# Autodesk Inventor assembly: 110033226_iam_07_中心城堡.iiam
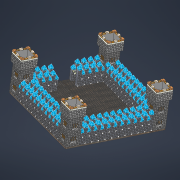
[picture p0: Inventor's stored thumbnail of the model, 180x180]
Saved by Autodesk Inventor 2022 (Build 260153000, 153)
## iProperties
Created: 2022-06-24
Part Number: 110033226_iam_07_中心城堡.iiam
Document SubType Name: Assembly
Designer: User
Author: User
## Documents named in this file (6)
- D:\D-disk\pomelo\大一\下學期\機械設計製圖\1100332260_LEGOproj_沒有公主城堡\110033226_iam_07_中心城堡.iiam.iam
- D:\D-disk\pomelo\大一\下學期\機械設計製圖\1100332260_LEGOproj_沒有公主城堡\110033226_ipt_33_中心城堡基座.ipt
- D:\D-disk\pomelo\大一\下學期\機械設計製圖\1100332260_LEGOproj_沒有公主城堡\110033226_iam_06_城堡四角塔.iam
- D:\D-disk\pomelo\大一\下學期\機械設計製圖\1100332260_LEGOproj_沒有公主城堡\110033226_ipt_34_中心城堡圍牆.ipt
- D:\D-disk\pomelo\大一\下學期\機械設計製圖\1100332260_LEGOproj_沒有公主城堡\110033226_ipt_34_中心城堡圍牆_MIR.ipt
- D:\D-disk\pomelo\大一\下學期\機械設計製圖\1100332260_LEGOproj_沒有公主城堡\110033226_ipt_35_中心城堡圍牆頂部_MIR.ipt
## Components (251 placed, 5 different names)
1. 110033226_ipt_33_中心城堡基座:1 — 貼合:1, 貼合:2, 貼合:3, 貼合:4, 貼合:5, 貼合:6, 貼合:7, 貼合:8, 貼合:9, 貼合:10, 貼合:11, 貼合:12, 貼合:24, 貼合:25, 貼合:26, 貼合:27, 貼合:29
2. 110033226_iam_06_城堡四角塔:1 [sub-assembly] — 貼合:4, 貼合:5, 貼合:6
3. 110033226_iam_06_城堡四角塔:2 [sub-assembly]
4. 110033226_iam_06_城堡四角塔:3 [sub-assembly]
5. 110033226_iam_06_城堡四角塔:4 [sub-assembly]
6. 110033226_ipt_34_中心城堡圍牆_MIR:1 — 貼合:10, 貼合:11, 貼合:12, 貼合:13, 貼合:14, 貼合:15, 貼合:16, 貼合:17
7. 110033226_ipt_34_中心城堡圍牆_MIR:2
8. 110033226_ipt_34_中心城堡圍牆_MIR:3
9. 110033226_ipt_34_中心城堡圍牆_MIR:4
10. 110033226_ipt_34_中心城堡圍牆_MIR:5
11. 110033226_ipt_34_中心城堡圍牆_MIR:6
12. 110033226_ipt_34_中心城堡圍牆_MIR:7
13. 110033226_ipt_34_中心城堡圍牆_MIR:8
14. 110033226_ipt_34_中心城堡圍牆_MIR:9
15. 110033226_ipt_34_中心城堡圍牆_MIR:10
16. 110033226_ipt_34_中心城堡圍牆_MIR:11
17. 110033226_ipt_34_中心城堡圍牆:1 — 貼合:7, 貼合:8, 貼合:9, 貼合:18, 貼合:19, 貼合:20, 貼合:21, 貼合:22, 貼合:23
18. 110033226_ipt_34_中心城堡圍牆:2
19. 110033226_ipt_34_中心城堡圍牆:3
20. 110033226_ipt_34_中心城堡圍牆:4
21. 110033226_ipt_34_中心城堡圍牆:5
22. 110033226_ipt_34_中心城堡圍牆:6
23. 110033226_ipt_34_中心城堡圍牆:7
24. 110033226_ipt_34_中心城堡圍牆:8
25. 110033226_ipt_34_中心城堡圍牆:9
26. 110033226_ipt_34_中心城堡圍牆:10
27. 110033226_ipt_34_中心城堡圍牆:11
28. 110033226_ipt_34_中心城堡圍牆_MIR:12
29. 110033226_ipt_34_中心城堡圍牆_MIR:13
30. 110033226_ipt_34_中心城堡圍牆_MIR:14
31. 110033226_ipt_34_中心城堡圍牆_MIR:15
32. 110033226_ipt_34_中心城堡圍牆_MIR:16
33. 110033226_ipt_34_中心城堡圍牆_MIR:17
34. 110033226_ipt_34_中心城堡圍牆_MIR:18
35. 110033226_ipt_34_中心城堡圍牆_MIR:19
36. 110033226_ipt_34_中心城堡圍牆_MIR:20
37. 110033226_ipt_34_中心城堡圍牆_MIR:21
38. 110033226_ipt_34_中心城堡圍牆_MIR:22
39. 110033226_ipt_34_中心城堡圍牆:12
40. 110033226_ipt_34_中心城堡圍牆:13
41. 110033226_ipt_34_中心城堡圍牆:14
42. 110033226_ipt_34_中心城堡圍牆:15
43. 110033226_ipt_34_中心城堡圍牆:16
44. 110033226_ipt_34_中心城堡圍牆:17
45. 110033226_ipt_34_中心城堡圍牆:18
46. 110033226_ipt_34_中心城堡圍牆:19
47. 110033226_ipt_34_中心城堡圍牆:20
48. 110033226_ipt_34_中心城堡圍牆:21
49. 110033226_ipt_34_中心城堡圍牆:22
50. 110033226_ipt_34_中心城堡圍牆_MIR:23
51. 110033226_ipt_34_中心城堡圍牆_MIR:24
52. 110033226_ipt_34_中心城堡圍牆_MIR:25
53. 110033226_ipt_34_中心城堡圍牆_MIR:26
54. 110033226_ipt_34_中心城堡圍牆_MIR:27
55. 110033226_ipt_34_中心城堡圍牆_MIR:28
56. 110033226_ipt_34_中心城堡圍牆_MIR:29
57. 110033226_ipt_34_中心城堡圍牆_MIR:30
58. 110033226_ipt_34_中心城堡圍牆_MIR:31
59. 110033226_ipt_34_中心城堡圍牆_MIR:32
60. 110033226_ipt_34_中心城堡圍牆_MIR:33
61. 110033226_ipt_34_中心城堡圍牆:23
62. 110033226_ipt_34_中心城堡圍牆:24
63. 110033226_ipt_34_中心城堡圍牆:25
64. 110033226_ipt_34_中心城堡圍牆:26
65. 110033226_ipt_34_中心城堡圍牆:27
66. 110033226_ipt_34_中心城堡圍牆:28
67. 110033226_ipt_34_中心城堡圍牆:29
68. 110033226_ipt_34_中心城堡圍牆:30
69. 110033226_ipt_34_中心城堡圍牆:31
70. 110033226_ipt_34_中心城堡圍牆:32
71. 110033226_ipt_34_中心城堡圍牆:33
72. 110033226_ipt_35_中心城堡圍牆頂部_MIR:3 — 貼合:16, 貼合:17
73. 110033226_ipt_35_中心城堡圍牆頂部_MIR:4 — 貼合:13, 貼合:14, 貼合:15
74. 110033226_ipt_35_中心城堡圍牆頂部_MIR:1 — 貼合:21, 貼合:22, 貼合:23
75. 110033226_ipt_35_中心城堡圍牆頂部_MIR:2 — 貼合:18, 貼合:19, 貼合:20
76. 110033226_ipt_35_中心城堡圍牆頂部_MIR:5
77. 110033226_ipt_35_中心城堡圍牆頂部_MIR:6
78. 110033226_ipt_35_中心城堡圍牆頂部_MIR:7
79. 110033226_ipt_35_中心城堡圍牆頂部_MIR:8
80. 110033226_ipt_35_中心城堡圍牆頂部_MIR:9
81. 110033226_ipt_35_中心城堡圍牆頂部_MIR:10
82. 110033226_ipt_35_中心城堡圍牆頂部_MIR:11
83. 110033226_ipt_35_中心城堡圍牆頂部_MIR:12
84. 110033226_ipt_35_中心城堡圍牆頂部_MIR:13
85. 110033226_ipt_35_中心城堡圍牆頂部_MIR:14
86. 110033226_ipt_35_中心城堡圍牆頂部_MIR:15
87. 110033226_ipt_35_中心城堡圍牆頂部_MIR:16
88. 110033226_ipt_35_中心城堡圍牆頂部_MIR:17
89. 110033226_ipt_35_中心城堡圍牆頂部_MIR:18
90. 110033226_ipt_35_中心城堡圍牆頂部_MIR:19
91. 110033226_ipt_35_中心城堡圍牆頂部_MIR:20
92. 110033226_ipt_35_中心城堡圍牆頂部_MIR:21
93. 110033226_ipt_35_中心城堡圍牆頂部_MIR:22
94. 110033226_ipt_35_中心城堡圍牆頂部_MIR:23
95. 110033226_ipt_35_中心城堡圍牆頂部_MIR:24
96. 110033226_ipt_35_中心城堡圍牆頂部_MIR:25
97. 110033226_ipt_35_中心城堡圍牆頂部_MIR:26
98. 110033226_ipt_35_中心城堡圍牆頂部_MIR:27
99. 110033226_ipt_35_中心城堡圍牆頂部_MIR:28
100. 110033226_ipt_35_中心城堡圍牆頂部_MIR:29
101. 110033226_ipt_35_中心城堡圍牆頂部_MIR:30
102. 110033226_ipt_35_中心城堡圍牆頂部_MIR:31
103. 110033226_ipt_35_中心城堡圍牆頂部_MIR:32
104. 110033226_ipt_35_中心城堡圍牆頂部_MIR:33
105. 110033226_ipt_35_中心城堡圍牆頂部_MIR:34
106. 110033226_ipt_35_中心城堡圍牆頂部_MIR:35
107. 110033226_ipt_35_中心城堡圍牆頂部_MIR:36
108. 110033226_ipt_35_中心城堡圍牆頂部_MIR:37
109. 110033226_ipt_35_中心城堡圍牆頂部_MIR:38
110. 110033226_ipt_35_中心城堡圍牆頂部_MIR:39
111. 110033226_ipt_35_中心城堡圍牆頂部_MIR:40
112. 110033226_ipt_35_中心城堡圍牆頂部_MIR:41
113. 110033226_ipt_35_中心城堡圍牆頂部_MIR:42
114. 110033226_ipt_35_中心城堡圍牆頂部_MIR:43
115. 110033226_ipt_35_中心城堡圍牆頂部_MIR:44
116. 110033226_ipt_35_中心城堡圍牆頂部_MIR:45
117. 110033226_ipt_35_中心城堡圍牆頂部_MIR:46
118. 110033226_ipt_35_中心城堡圍牆頂部_MIR:47
119. 110033226_ipt_35_中心城堡圍牆頂部_MIR:48
120. 110033226_ipt_35_中心城堡圍牆頂部_MIR:49
121. 110033226_ipt_35_中心城堡圍牆頂部_MIR:50
122. 110033226_ipt_35_中心城堡圍牆頂部_MIR:51
123. 110033226_ipt_35_中心城堡圍牆頂部_MIR:52
124. 110033226_ipt_35_中心城堡圍牆頂部_MIR:53
125. 110033226_ipt_35_中心城堡圍牆頂部_MIR:54
126. 110033226_ipt_35_中心城堡圍牆頂部_MIR:55
127. 110033226_ipt_35_中心城堡圍牆頂部_MIR:56
128. 110033226_ipt_35_中心城堡圍牆頂部_MIR:57
129. 110033226_ipt_35_中心城堡圍牆頂部_MIR:58
130. 110033226_ipt_35_中心城堡圍牆頂部_MIR:59
131. 110033226_ipt_35_中心城堡圍牆頂部_MIR:60
132. 110033226_ipt_35_中心城堡圍牆頂部_MIR:61
133. 110033226_ipt_35_中心城堡圍牆頂部_MIR:62
134. 110033226_ipt_35_中心城堡圍牆頂部_MIR:63
135. 110033226_ipt_35_中心城堡圍牆頂部_MIR:64
136. 110033226_ipt_35_中心城堡圍牆頂部_MIR:65
137. 110033226_ipt_35_中心城堡圍牆頂部_MIR:66
138. 110033226_ipt_35_中心城堡圍牆頂部_MIR:67
139. 110033226_ipt_35_中心城堡圍牆頂部_MIR:68
140. 110033226_ipt_35_中心城堡圍牆頂部_MIR:69
141. 110033226_ipt_35_中心城堡圍牆頂部_MIR:70
142. 110033226_ipt_35_中心城堡圍牆頂部_MIR:71
143. 110033226_ipt_35_中心城堡圍牆頂部_MIR:72
144. 110033226_ipt_35_中心城堡圍牆頂部_MIR:73
145. 110033226_ipt_35_中心城堡圍牆頂部_MIR:74
146. 110033226_ipt_35_中心城堡圍牆頂部_MIR:75
147. 110033226_ipt_35_中心城堡圍牆頂部_MIR:76
148. 110033226_ipt_35_中心城堡圍牆頂部_MIR:77
149. 110033226_ipt_35_中心城堡圍牆頂部_MIR:78
150. 110033226_ipt_35_中心城堡圍牆頂部_MIR:79
151. 110033226_ipt_35_中心城堡圍牆頂部_MIR:80
152. 110033226_ipt_35_中心城堡圍牆頂部_MIR:81
153. 110033226_ipt_35_中心城堡圍牆頂部_MIR:82
154. 110033226_ipt_35_中心城堡圍牆頂部_MIR:83
155. 110033226_ipt_35_中心城堡圍牆頂部_MIR:84
156. 110033226_ipt_35_中心城堡圍牆頂部_MIR:85
157. 110033226_ipt_35_中心城堡圍牆頂部_MIR:86
158. 110033226_ipt_35_中心城堡圍牆頂部_MIR:87
159. 110033226_ipt_35_中心城堡圍牆頂部_MIR:88
160. 110033226_ipt_35_中心城堡圍牆頂部_MIR:89
161. 110033226_ipt_35_中心城堡圍牆頂部_MIR:90
162. 110033226_ipt_35_中心城堡圍牆頂部_MIR:91
163. 110033226_ipt_35_中心城堡圍牆頂部_MIR:92
164. 110033226_ipt_35_中心城堡圍牆頂部_MIR:93
165. 110033226_ipt_35_中心城堡圍牆頂部_MIR:94
166. 110033226_ipt_35_中心城堡圍牆頂部_MIR:95
167. 110033226_ipt_35_中心城堡圍牆頂部_MIR:96
168. 110033226_ipt_35_中心城堡圍牆頂部_MIR:97
169. 110033226_ipt_35_中心城堡圍牆頂部_MIR:98
170. 110033226_ipt_35_中心城堡圍牆頂部_MIR:99
171. 110033226_ipt_35_中心城堡圍牆頂部_MIR:100
172. 110033226_ipt_35_中心城堡圍牆頂部_MIR:101
173. 110033226_ipt_35_中心城堡圍牆頂部_MIR:102
174. 110033226_ipt_35_中心城堡圍牆頂部_MIR:103
175. 110033226_ipt_35_中心城堡圍牆頂部_MIR:104
176. 110033226_ipt_35_中心城堡圍牆頂部_MIR:105
177. 110033226_ipt_35_中心城堡圍牆頂部_MIR:106
178. 110033226_ipt_35_中心城堡圍牆頂部_MIR:107
179. 110033226_ipt_35_中心城堡圍牆頂部_MIR:108
180. 110033226_ipt_35_中心城堡圍牆頂部_MIR:109
181. 110033226_ipt_35_中心城堡圍牆頂部_MIR:110
182. 110033226_ipt_35_中心城堡圍牆頂部_MIR:111
183. 110033226_ipt_35_中心城堡圍牆頂部_MIR:112
184. 110033226_ipt_35_中心城堡圍牆頂部_MIR:113
185. 110033226_ipt_35_中心城堡圍牆頂部_MIR:114
186. 110033226_ipt_35_中心城堡圍牆頂部_MIR:115
187. 110033226_ipt_35_中心城堡圍牆頂部_MIR:116
188. 110033226_ipt_35_中心城堡圍牆頂部_MIR:117
189. 110033226_ipt_35_中心城堡圍牆頂部_MIR:118
190. 110033226_ipt_35_中心城堡圍牆頂部_MIR:119
191. 110033226_ipt_35_中心城堡圍牆頂部_MIR:120
192. 110033226_ipt_35_中心城堡圍牆頂部_MIR:121
193. 110033226_ipt_35_中心城堡圍牆頂部_MIR:122
194. 110033226_ipt_35_中心城堡圍牆頂部_MIR:123
195. 110033226_ipt_35_中心城堡圍牆頂部_MIR:124
196. 110033226_ipt_35_中心城堡圍牆頂部_MIR:125
197. 110033226_ipt_35_中心城堡圍牆頂部_MIR:126
198. 110033226_ipt_35_中心城堡圍牆頂部_MIR:127
199. 110033226_ipt_35_中心城堡圍牆頂部_MIR:128
200. 110033226_ipt_35_中心城堡圍牆頂部_MIR:129
201. 110033226_ipt_35_中心城堡圍牆頂部_MIR:130
202. 110033226_ipt_35_中心城堡圍牆頂部_MIR:131
203. 110033226_ipt_35_中心城堡圍牆頂部_MIR:132
204. 110033226_ipt_34_中心城堡圍牆_MIR:34 — 貼合:24, 貼合:25, 貼合:26, 貼合:28, 貼合:30, 貼合:31, 貼合:32, 貼合:39, 貼合:40, 貼合:41
205. 110033226_ipt_34_中心城堡圍牆_MIR:35 — 貼合:27, 貼合:28, 貼合:29, 貼合:33, 貼合:34, 貼合:35, 貼合:36, 貼合:37, 貼合:38
206. 110033226_ipt_34_中心城堡圍牆_MIR:36
207. 110033226_ipt_34_中心城堡圍牆_MIR:37
208. 110033226_ipt_34_中心城堡圍牆_MIR:38
209. 110033226_ipt_34_中心城堡圍牆_MIR:39
210. 110033226_ipt_34_中心城堡圍牆_MIR:40
211. 110033226_ipt_34_中心城堡圍牆_MIR:41
212. 110033226_ipt_34_中心城堡圍牆_MIR:42
213. 110033226_ipt_34_中心城堡圍牆_MIR:43
214. 110033226_ipt_34_中心城堡圍牆_MIR:44
215. 110033226_ipt_34_中心城堡圍牆_MIR:45
216. 110033226_ipt_34_中心城堡圍牆_MIR:46
217. 110033226_ipt_34_中心城堡圍牆_MIR:47
218. 110033226_ipt_34_中心城堡圍牆_MIR:48
219. 110033226_ipt_34_中心城堡圍牆_MIR:49
220. 110033226_ipt_35_中心城堡圍牆頂部_MIR:134 — 貼合:33, 貼合:34, 貼合:35
221. 110033226_ipt_35_中心城堡圍牆頂部_MIR:136 — 貼合:36, 貼合:37, 貼合:38
222. 110033226_ipt_35_中心城堡圍牆頂部_MIR:133 — 貼合:30, 貼合:31, 貼合:32
223. 110033226_ipt_35_中心城堡圍牆頂部_MIR:135 — 貼合:39, 貼合:40, 貼合:41
224. 110033226_ipt_35_中心城堡圍牆頂部_MIR:137
225. 110033226_ipt_35_中心城堡圍牆頂部_MIR:138
226. 110033226_ipt_35_中心城堡圍牆頂部_MIR:139
227. 110033226_ipt_35_中心城堡圍牆頂部_MIR:140
228. 110033226_ipt_35_中心城堡圍牆頂部_MIR:141
229. 110033226_ipt_35_中心城堡圍牆頂部_MIR:142
230. 110033226_ipt_35_中心城堡圍牆頂部_MIR:143
231. 110033226_ipt_35_中心城堡圍牆頂部_MIR:144
232. 110033226_ipt_35_中心城堡圍牆頂部_MIR:145
233. 110033226_ipt_35_中心城堡圍牆頂部_MIR:146
234. 110033226_ipt_35_中心城堡圍牆頂部_MIR:147
235. 110033226_ipt_35_中心城堡圍牆頂部_MIR:148
236. 110033226_ipt_35_中心城堡圍牆頂部_MIR:149
237. 110033226_ipt_35_中心城堡圍牆頂部_MIR:150
238. 110033226_ipt_35_中心城堡圍牆頂部_MIR:151
239. 110033226_ipt_35_中心城堡圍牆頂部_MIR:152
240. 110033226_ipt_35_中心城堡圍牆頂部_MIR:153
241. 110033226_ipt_35_中心城堡圍牆頂部_MIR:154
242. 110033226_ipt_35_中心城堡圍牆頂部_MIR:155
243. 110033226_ipt_35_中心城堡圍牆頂部_MIR:156
244. 110033226_ipt_35_中心城堡圍牆頂部_MIR:157
245. 110033226_ipt_35_中心城堡圍牆頂部_MIR:158
246. 110033226_ipt_35_中心城堡圍牆頂部_MIR:159
247. 110033226_ipt_35_中心城堡圍牆頂部_MIR:160
248. 110033226_ipt_35_中心城堡圍牆頂部_MIR:161
249. 110033226_ipt_35_中心城堡圍牆頂部_MIR:162
250. 110033226_ipt_35_中心城堡圍牆頂部_MIR:163
251. 110033226_ipt_35_中心城堡圍牆頂部_MIR:164
## Component patterns: (4 elements, first: 110033226_iam_06_城堡四角塔:1), (3 elements), (3 elements), (2 elements), (2 elements), (11 elements, first: 110033226_ipt_34_中心城堡圍牆_MIR:1), (11 elements, first: 110033226_ipt_34_中心城堡圍牆:1), 元件陣列 7:2 (11 elements), 元件陣列 4:2 (11 elements), 元件陣列 7:3 (11 elements), 元件陣列 4:3 (11 elements), (11 elements, first: 110033226_ipt_35_中心城堡圍牆頂部_MIR:3 + 110033226_ipt_35_中心城堡圍牆頂部_MIR:4 + 110033226_ipt_35_中心城堡圍牆頂部_MIR:1 + 110033226_ipt_35_中心城堡圍牆頂部_MIR:2), 元件陣列 9:2 (11 elements), 元件陣列 9:3 (11 elements), (4 elements, first: 110033226_ipt_34_中心城堡圍牆_MIR:34 + 110033226_ipt_34_中心城堡圍牆_MIR:35), 元件陣列 11:2 (4 elements), (4 elements, first: 110033226_ipt_35_中心城堡圍牆頂部_MIR:134 + 110033226_ipt_35_中心城堡圍牆頂部_MIR:136 + 110033226_ipt_35_中心城堡圍牆頂部_MIR:133 + 110033226_ipt_35_中心城堡圍牆頂部_MIR:135), 元件陣列 13:2 (4 elements)
## Relationships (41: Mate 41)
- 貼合:1 [Mate]: 110033226_ipt_33_中心城堡基座:1
- 貼合:2 [Mate]: 110033226_ipt_33_中心城堡基座:1
- 貼合:3 [Mate]: 110033226_ipt_33_中心城堡基座:1
- 貼合:4 [Mate]: 110033226_ipt_33_中心城堡基座:1 ↔ 110033226_iam_06_城堡四角塔:1
- 貼合:5 [Mate]: 110033226_ipt_33_中心城堡基座:1 ↔ 110033226_iam_06_城堡四角塔:1
- 貼合:6 [Mate]: 110033226_ipt_33_中心城堡基座:1 ↔ 110033226_iam_06_城堡四角塔:1
- 貼合:7 [Mate]: 110033226_ipt_33_中心城堡基座:1 ↔ 110033226_ipt_34_中心城堡圍牆:1
- 貼合:8 [Mate]: 110033226_ipt_33_中心城堡基座:1 ↔ 110033226_ipt_34_中心城堡圍牆:1
- 貼合:9 [Mate]: 110033226_ipt_33_中心城堡基座:1 ↔ 110033226_ipt_34_中心城堡圍牆:1
- 貼合:10 [Mate]: 110033226_ipt_33_中心城堡基座:1 ↔ 110033226_ipt_34_中心城堡圍牆_MIR:1
- 貼合:11 [Mate]: 110033226_ipt_33_中心城堡基座:1 ↔ 110033226_ipt_34_中心城堡圍牆_MIR:1
- 貼合:12 [Mate]: 110033226_ipt_33_中心城堡基座:1 ↔ 110033226_ipt_34_中心城堡圍牆_MIR:1
- 貼合:13 [Mate]: 110033226_ipt_34_中心城堡圍牆_MIR:1 ↔ 110033226_ipt_35_中心城堡圍牆頂部_MIR:4
- 貼合:14 [Mate]: 110033226_ipt_34_中心城堡圍牆_MIR:1 ↔ 110033226_ipt_35_中心城堡圍牆頂部_MIR:4
- 貼合:15 [Mate]: 110033226_ipt_34_中心城堡圍牆_MIR:1 ↔ 110033226_ipt_35_中心城堡圍牆頂部_MIR:4
- 貼合:16 [Mate]: 110033226_ipt_34_中心城堡圍牆_MIR:1 ↔ 110033226_ipt_35_中心城堡圍牆頂部_MIR:3
- 貼合:17 [Mate]: 110033226_ipt_34_中心城堡圍牆_MIR:1 ↔ 110033226_ipt_35_中心城堡圍牆頂部_MIR:3
- 貼合:18 [Mate]: 110033226_ipt_34_中心城堡圍牆:1 ↔ 110033226_ipt_35_中心城堡圍牆頂部_MIR:2
- 貼合:19 [Mate]: 110033226_ipt_34_中心城堡圍牆:1 ↔ 110033226_ipt_35_中心城堡圍牆頂部_MIR:2
- 貼合:20 [Mate]: 110033226_ipt_34_中心城堡圍牆:1 ↔ 110033226_ipt_35_中心城堡圍牆頂部_MIR:2
- 貼合:21 [Mate]: 110033226_ipt_34_中心城堡圍牆:1 ↔ 110033226_ipt_35_中心城堡圍牆頂部_MIR:1
- 貼合:22 [Mate]: 110033226_ipt_34_中心城堡圍牆:1 ↔ 110033226_ipt_35_中心城堡圍牆頂部_MIR:1
- 貼合:23 [Mate]: 110033226_ipt_34_中心城堡圍牆:1 ↔ 110033226_ipt_35_中心城堡圍牆頂部_MIR:1
- 貼合:24 [Mate]: 110033226_ipt_33_中心城堡基座:1 ↔ 110033226_ipt_34_中心城堡圍牆_MIR:34
- 貼合:25 [Mate]: 110033226_ipt_33_中心城堡基座:1 ↔ 110033226_ipt_34_中心城堡圍牆_MIR:34
- 貼合:26 [Mate]: 110033226_ipt_33_中心城堡基座:1 ↔ 110033226_ipt_34_中心城堡圍牆_MIR:34
- 貼合:27 [Mate]: 110033226_ipt_33_中心城堡基座:1 ↔ 110033226_ipt_34_中心城堡圍牆_MIR:35
- 貼合:28 [Mate]: 110033226_ipt_34_中心城堡圍牆_MIR:34 ↔ 110033226_ipt_34_中心城堡圍牆_MIR:35
- 貼合:29 [Mate]: 110033226_ipt_33_中心城堡基座:1 ↔ 110033226_ipt_34_中心城堡圍牆_MIR:35
- 貼合:30 [Mate]: 110033226_ipt_34_中心城堡圍牆_MIR:34 ↔ 110033226_ipt_35_中心城堡圍牆頂部_MIR:133
- 貼合:31 [Mate]: 110033226_ipt_34_中心城堡圍牆_MIR:34 ↔ 110033226_ipt_35_中心城堡圍牆頂部_MIR:133
- 貼合:32 [Mate]: 110033226_ipt_34_中心城堡圍牆_MIR:34 ↔ 110033226_ipt_35_中心城堡圍牆頂部_MIR:133
- 貼合:33 [Mate]: 110033226_ipt_34_中心城堡圍牆_MIR:35 ↔ 110033226_ipt_35_中心城堡圍牆頂部_MIR:134
- 貼合:34 [Mate]: 110033226_ipt_34_中心城堡圍牆_MIR:35 ↔ 110033226_ipt_35_中心城堡圍牆頂部_MIR:134
- 貼合:35 [Mate]: 110033226_ipt_34_中心城堡圍牆_MIR:35 ↔ 110033226_ipt_35_中心城堡圍牆頂部_MIR:134
- 貼合:36 [Mate]: 110033226_ipt_34_中心城堡圍牆_MIR:35 ↔ 110033226_ipt_35_中心城堡圍牆頂部_MIR:136
- 貼合:37 [Mate]: 110033226_ipt_34_中心城堡圍牆_MIR:35 ↔ 110033226_ipt_35_中心城堡圍牆頂部_MIR:136
- 貼合:38 [Mate]: 110033226_ipt_34_中心城堡圍牆_MIR:35 ↔ 110033226_ipt_35_中心城堡圍牆頂部_MIR:136
- 貼合:39 [Mate]: 110033226_ipt_34_中心城堡圍牆_MIR:34 ↔ 110033226_ipt_35_中心城堡圍牆頂部_MIR:135
- 貼合:40 [Mate]: 110033226_ipt_34_中心城堡圍牆_MIR:34 ↔ 110033226_ipt_35_中心城堡圍牆頂部_MIR:135
- 貼合:41 [Mate]: 110033226_ipt_34_中心城堡圍牆_MIR:34 ↔ 110033226_ipt_35_中心城堡圍牆頂部_MIR:135
